# Autodesk Inventor assembly: parachute_structure_asm
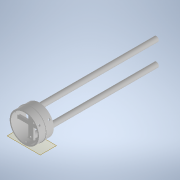
[picture p0: Inventor's stored thumbnail of the model, 180x180]
Saved by Autodesk Inventor 2020 (Build 240168000, 168)
## iProperties
Created: 2022-03-10
Part Number: parachute_structure_asm
Document SubType Name: Assembly
Designer: sp
Author: sp
## Documents named in this file (3)
- C:\Users\sp\Documents\Rocket\rocket\CAD\parachute_structure_asm.iam
- C:\Users\sp\Documents\Rocket\rocket\CAD\stange.ipt
- C:\Users\sp\Documents\Rocket\rocket\CAD\Verbindungsring_2_2.ipt
## Components (3 placed, 2 different names)
1. stange:1 — Einfügen:1
2. stange:2 — Einfügen:2
3. Verbindungsring_2_2:1 — Einfügen:1, Einfügen:2
## Relationships (2: Insert 2)
- Einfügen:1 [Insert]: stange:1 ↔ Verbindungsring_2_2:1
- Einfügen:2 [Insert]: stange:2 ↔ Verbindungsring_2_2:1
